# Autodesk Inventor assembly: plog-blade-hold
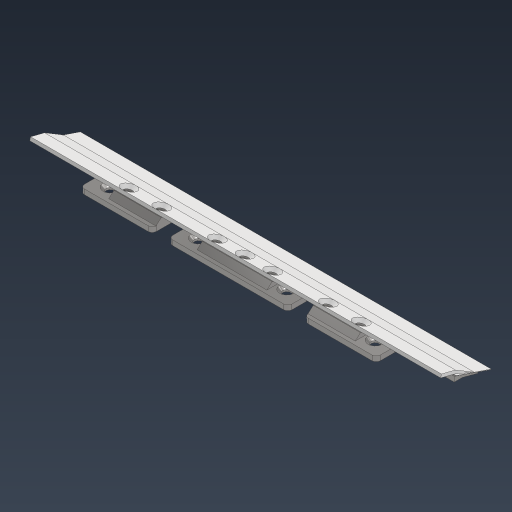
[picture p0: Inventor's stored thumbnail of the model, 512x512]
Saved by Autodesk Inventor 2023 (Build 270158000, 158)
## iProperties
Created: 2025-10-16
Part Number: plog-blade-hold
Document SubType Name: Assembly
Designer: szymo
Author: szymo
## Documents named in this file (5)
- D:\tech\robotyka\robots\codename wafel - australia\3d_parts\rev4\plog-blade-hold.iam
- D:\tech\robotyka\robots\codename wafel - australia\3d_parts\rev4\plog.ipt
- D:\tech\robotyka\robots\codename wafel - australia\3d_parts\rev4\blade.ipt
- D:\tech\robotyka\robots\codename wafel - australia\3d_parts\rev4\blade-hold.ipt
- D:\tech\robotyka\robots\codename wafel - australia\3d_parts\rev4\blade-uphold.ipt
## Components (4 placed, 4 different names)
1. blade-hold:1 — Flush:2, Flush:3, Flush:4, Flush:5
2. plog:1 — Flush:1, Mate:1, Mate:2, Flush:2, Flush:3, Flush:4
3. blade:1 — Flush:1, Mate:1, Mate:2
4. blade-uphold:1 — Flush:5
## Relationships (7: Flush 5, Mate 2)
- Flush:1 (10 mm): plog:1 ↔ blade:1
- Mate:1: plog:1 ↔ blade:1
- Mate:2 (1 mm): plog:1 ↔ blade:1
- Flush:2: blade-hold:1 ↔ plog:1
- Flush:3: blade-hold:1 ↔ plog:1
- Flush:4: blade-hold:1 ↔ plog:1
- Flush:5: blade-hold:1 ↔ blade-uphold:1
